# Autodesk Inventor assembly: 200-30-BOGIE-BEARING-ASM-01
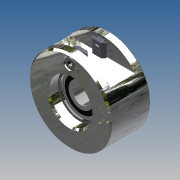
[picture p0: Inventor's stored thumbnail of the model, 180x180]
Saved by Autodesk Inventor 2018.2 (Build 222227000, 227)
## iProperties
Manager: feesmrt
Company: FRANC0R
Created: 2017-12-10
Part Number: 200-30-BOGIE-BEARING-ASM-01
Material: Generisch
Document SubType Name: Assembly
Designer: feesmrt
Project: Rescue Robot
Cost Center: -
Description: Bogie Bearing Assembly
Engineer: feesmrt
Authority: feesmrt
Stock Number: 200-30-BOGIE-BEARING-ASM-01
Author: feesmrt
Title: Bogie Bearing Assembly
Subject: Rescue Robot
Revision Number: 1
## Documents named in this file (6)
- D:\Programmierung\FRANC0R\CAD\02-Rocker-Bogie-Robot\200-ROCKER-BOGIE\200-30-BOGIE-BEARING\200-30-BOGIE-BEARING-ASM-01.iam
- D:\Programmierung\FRANC0R\CAD\02-Rocker-Bogie-Robot\200-ROCKER-BOGIE\200-30-BOGIE-BEARING\200-30-ROCKER-BOGIE-BEARING-01.ipt
- D:\Programmierung\FRANC0R\CAD\02-Rocker-Bogie-Robot\900-COMPONENTS\900-20-BEARINGS\900-20-BEARINGS-3304-2RS-TN.ipt
- D:\Programmierung\FRANC0R\CAD\02-Rocker-Bogie-Robot\900-COMPONENTS\900-60-CIRCLIPS\900-60-CIRCLIPS-DIN472-52x2.ipt
- D:\Programmierung\FRANC0R\CAD\02-Rocker-Bogie-Robot\900-COMPONENTS\900-50-PROFILES\900-50-PROFILES-CONN-N8xM8.ipt
- D:\Programmierung\FRANC0R\CAD\02-Rocker-Bogie-Robot\900-COMPONENTS\900-40-SCREWS\900-40-SCREWS-DIN7984_M8x12.ipt
## Components (7 placed, 5 different names)
1. 200-30-ROCKER-BOGIE-BEARING-01:1 — Passend:1, Passend:2, Passend:3, Passend:4, Passend:5, Passend:6, Passend:7, Passend:8, Winkel:1, Winkel:2, Passend:9, Passend:11, Passend:12
2. 900-20-BEARINGS-3304-2RS-TN:1 — Passend:1, Passend:2
3. 900-60-CIRCLIPS-DIN472-52x2:1 — Passend:3, Passend:4
4. 900-50-PROFILES-CONN-N8xM8:1 — Passend:5, Passend:7, Winkel:1, Passend:10
5. 900-50-PROFILES-CONN-N8xM8:2 — Passend:6, Passend:8, Winkel:2
6. 900-40-SCREWS-DIN7984_M8x12:1 — Passend:9, Passend:11
7. 900-40-SCREWS-DIN7984_M8x12:2 — Passend:10, Passend:12
## Relationships (14: Mate 12, Angle 2)
- Passend:1 [Mate]: 200-30-ROCKER-BOGIE-BEARING-01:1 ↔ 900-20-BEARINGS-3304-2RS-TN:1
- Passend:2 [Mate]: 200-30-ROCKER-BOGIE-BEARING-01:1 ↔ 900-20-BEARINGS-3304-2RS-TN:1
- Passend:3 [Mate]: 200-30-ROCKER-BOGIE-BEARING-01:1 ↔ 900-60-CIRCLIPS-DIN472-52x2:1
- Passend:4 [Mate]: 200-30-ROCKER-BOGIE-BEARING-01:1 ↔ 900-60-CIRCLIPS-DIN472-52x2:1
- Passend:5 [Mate]: 200-30-ROCKER-BOGIE-BEARING-01:1 ↔ 900-50-PROFILES-CONN-N8xM8:1
- Passend:6 [Mate]: 200-30-ROCKER-BOGIE-BEARING-01:1 ↔ 900-50-PROFILES-CONN-N8xM8:2
- Passend:7 [Mate] (2.8 mm): 200-30-ROCKER-BOGIE-BEARING-01:1 ↔ 900-50-PROFILES-CONN-N8xM8:1
- Passend:8 [Mate] (2.8 mm): 200-30-ROCKER-BOGIE-BEARING-01:1 ↔ 900-50-PROFILES-CONN-N8xM8:2
- Winkel:1 [Angle] (0 deg): 200-30-ROCKER-BOGIE-BEARING-01:1 ↔ 900-50-PROFILES-CONN-N8xM8:1
- Winkel:2 [Angle] (0 deg): 200-30-ROCKER-BOGIE-BEARING-01:1 ↔ 900-50-PROFILES-CONN-N8xM8:2
- Passend:9 [Mate]: 200-30-ROCKER-BOGIE-BEARING-01:1 ↔ 900-40-SCREWS-DIN7984_M8x12:1
- Passend:10 [Mate]: 900-50-PROFILES-CONN-N8xM8:1 ↔ 900-40-SCREWS-DIN7984_M8x12:2
- Passend:11 [Mate]: 200-30-ROCKER-BOGIE-BEARING-01:1 ↔ 900-40-SCREWS-DIN7984_M8x12:1
- Passend:12 [Mate]: 200-30-ROCKER-BOGIE-BEARING-01:1 ↔ 900-40-SCREWS-DIN7984_M8x12:2
